# Autodesk Inventor assembly: Cockpit
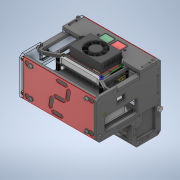
[picture p0: Inventor's stored thumbnail of the model, 180x180]
Saved by Autodesk Inventor 2022.3 (Build 263350000, 350)
## iProperties
Created: 2022-04-25
Part Number: Cockpit
Document SubType Name: Assembly
Designer: Masato Kubotera
Author: Masato Kubotera
## Documents named in this file (26)
- C:\Users\Masato\Documents\Inventor\Inventor for CIT Brains\SUSTAINA-OP - Cockpit mate\UpperBody\Cockpit\Cockpit.iam
- C:\Users\Masato\Documents\Inventor\Inventor for CIT Brains\SUSTAINA-OP - Cockpit mate\UpperBody\Cockpit\Cockpit_side_frame_MIR.ipt
- C:\Users\Masato\Documents\Inventor\Inventor for CIT Brains\SUSTAINA-OP - Cockpit mate\UpperBody\Cockpit\Cockpit_circuit_board_frame.ipt
- C:\Users\Masato\Documents\Inventor\Inventor for CIT Brains\SUSTAINA-OP - Cockpit mate\UpperBody\Cockpit\Cockpit_battery_back_door.ipt
- C:\Users\Masato\Documents\Inventor\Inventor for CIT Brains\SUSTAINA-OP - Cockpit mate\UpperBody\Cockpit\Cockpit_side_frame.ipt
- C:\Users\Masato\Documents\Inventor\Inventor for CIT Brains\SUSTAINA-OP - Cockpit mate\ReadyMade\InsertNut\IRU-304S.ipt
- C:\Users\Masato\Documents\Inventor\Inventor for CIT Brains\SUSTAINA-OP - Cockpit mate\ReadyMade\InsertNut\UD-43040.ipt
- C:\Users\Masato\Documents\Inventor\Inventor for CIT Brains\SUSTAINA-OP - Cockpit mate\ReadyMade\Neodymium_magnet_Phi3_T3.ipt
- C:\Users\Masato\Documents\Inventor\Inventor for CIT Brains\SUSTAINA-OP - Cockpit mate\UpperBody\Cockpit\Cockpit_front_frame_cloth.ipt
- C:\Users\Masato\Documents\Inventor\Inventor for CIT Brains\SUSTAINA-OP - Cockpit mate\UpperBody\Cockpit\Cockpit_back_frame_cloth.ipt
- C:\Users\Masato\Documents\Inventor\Inventor for CIT Brains\SUSTAINA-OP - Cockpit mate\ElectronicComponents\Board_designed_for_SUSTAINA-OP\SUSTAINA-Core-Board.ipt
- C:\Users\Masato\Documents\Inventor\Inventor for CIT Brains\SUSTAINA-OP - Cockpit mate\UpperBody\Cockpit\MainBoard_cover.ipt
- C:\Users\Masato\Documents\Inventor\Inventor for CIT Brains\SUSTAINA-OP - Cockpit mate\ReadyMade\Battery\HP-G830C2800S3.ipt
- C:\Users\Masato\Documents\Inventor\Inventor for CIT Brains\SUSTAINA-OP - Cockpit mate\ReadyMade\Screw\UC-0306.ipt
- C:\Users\Masato\Documents\Inventor\Inventor for CIT Brains\SUSTAINA-OP - Cockpit mate\ReadyMade\Screw\UC-0308.ipt
- C:\Users\Masato\Documents\Inventor\Inventor for CIT Brains\SUSTAINA-OP - Cockpit mate\ElectronicComponents\Board_designed_for_SUSTAINA-OP\Control-Buttons-Module.ipt
- C:\Users\Masato\Documents\Inventor\Inventor for CIT Brains\SUSTAINA-OP - Cockpit mate\ReadyMade\Screw\SPNFL-BRN-M3-10.ipt
- C:\Users\Masato\Documents\Inventor\Inventor for CIT Brains\SUSTAINA-OP - Cockpit mate\UpperBody\Cockpit\Cockpit_carrier_board_frame.iam
- C:\Users\Masato\Documents\Inventor\Inventor for CIT Brains\SUSTAINA-OP - Cockpit mate\UpperBody\Cockpit\Cockpit_top_frame.iam
- C:\Users\Masato\Documents\Inventor\Inventor for CIT Brains\SUSTAINA-OP - Cockpit mate\ElectronicComponents\SingleBoardComputerUnit.iam
- C:\Users\Masato\Documents\Inventor\Inventor for CIT Brains\SUSTAINA-OP - Cockpit mate\UpperBody\Cockpit\Cockpit_from_frame.iam
- C:\Users\Masato\Documents\Inventor\Inventor for CIT Brains\SUSTAINA-OP - Cockpit mate\ReadyMade\Bush\L3040-8110TB.ipt
- C:\Users\Masato\Documents\Inventor\Inventor for CIT Brains\SUSTAINA-OP - Cockpit mate\UpperBody\Cockpit\Cockpit_back_frame.iam
- C:\Users\Masato\Documents\Inventor\Inventor for CIT Brains\SUSTAINA-OP - Cockpit mate\ReadyMade\Screw\UC-2610.ipt
- C:\Users\Masato\Documents\Inventor\Inventor for CIT Brains\SUSTAINA-OP - Cockpit mate\ReadyMade\Spacer\BRU-305.ipt
- C:\Users\Masato\Documents\Inventor\Inventor for CIT Brains\SUSTAINA-OP - Cockpit mate\UpperBody\Cockpit\Cockpit_battery_frame.iam
## Components (88 placed, 25 different names)
1. SUSTAINA-Core-Board:1 — 挿入:63, 挿入:64, 挿入:65, 挿入:66, 挿入:95, 挿入:96, 挿入:166, 挿入:167
2. Control-Buttons-Module:1 — 挿入:105, 挿入:106, 挿入:138, 挿入:139
3. Cockpit_carrier_board_frame:1 [sub-assembly] — 挿入:140, 挿入:141, 挿入:144, 挿入:145, 挿入:149
4. Cockpit_carrier_board_frame:2 [sub-assembly] — 挿入:142, 挿入:143, 挿入:146, 挿入:147
5. Cockpit_top_frame:1 [sub-assembly] — 挿入:138, 挿入:139, 挿入:150, 挿入:151, 挿入:152, 挿入:153
6. SingleBoardComputerUnit:1 [sub-assembly] — 挿入:140, 挿入:141, 挿入:142, 挿入:143
7. UC-0308:13 — 挿入:146
8. UC-0308:14 — 挿入:147
9. Cockpit_from_frame:1 [sub-assembly] — 挿入:154, 挿入:155, 挿入:156, 挿入:157, 挿入:158, 挿入:159, 挿入:165
10. L3040-8110TB:1 — 挿入:156, 挿入:160, 挿入:164
11. L3040-8110TB:2 — 挿入:157, 挿入:161
12. L3040-8110TB:3 — 挿入:158, 挿入:162
13. L3040-8110TB:4 — 挿入:159, 挿入:163
14. UC-0306:25 — 挿入:160
15. UC-0306:26 — 挿入:161
16. UC-0306:27 — 挿入:162
17. UC-0306:28 — 挿入:163
18. UC-0308:15 — 挿入:166
19. UC-0308:16 — 挿入:167
20. Cockpit_back_frame:1 [sub-assembly] — 挿入:168, 挿入:169, 挿入:174, 挿入:175, 挿入:176, 挿入:177, 挿入:180, 挿入:181
21. L3040-8110TB:5 — 挿入:174, 挿入:178
22. UC-0306:29
23. L3040-8110TB:6 — 挿入:175, 挿入:179
24. UC-0306:30
25. L3040-8110TB:7 — 挿入:176
26. UC-0306:31
27. L3040-8110TB:8 — 挿入:177
28. UC-0306:32
29. UC-2610:1 — 挿入:180
30. UC-2610:2 — 挿入:181
31. BRU-305:1 — 挿入:182
32. BRU-305:2 — 挿入:183
33. Cockpit_battery_frame:1 [sub-assembly] — 挿入:184, 角度:4
34. Cockpit_battery_frame:2 [sub-assembly] — 挿入:185, 角度:5
35. Cockpit_side_frame_MIR:1 — 挿入:12, 挿入:23, 挿入:42, 挿入:46, 挿入:47, 挿入:48, 挿入:75, 挿入:77, 挿入:79, 挿入:80, 挿入:81, 挿入:82, 挿入:134, 挿入:137, 挿入:183
36. Cockpit_circuit_board_frame:1 — メイト:3, メイト:4, フラッシュ:8, 挿入:55, 挿入:56, 挿入:57, 挿入:58
37. Cockpit_battery_back_door:1 — 挿入:41, 挿入:42, 挿入:49, 挿入:50, 挿入:51, 挿入:52, 挿入:53, 挿入:54, 角度:3
38. Cockpit_side_frame:1 — フラッシュ:1, フラッシュ:2, フラッシュ:3, 挿入:10, 挿入:21, 挿入:41, 挿入:43, 挿入:44, 挿入:45, メイト:3, メイト:4, フラッシュ:8, 挿入:67, 挿入:68, 挿入:69, 挿入:71, 挿入:72, 挿入:73, 挿入:74, 挿入:133, 角度:3, 挿入:149, 挿入:154, 挿入:155, 挿入:168, 挿入:169, 挿入:182, 挿入:184, 角度:4, 挿入:185, 角度:5
39. Cockpit_front_frame_cloth:1 — 挿入:164, 挿入:165
40. Cockpit_back_frame_cloth:1 — 挿入:178, 挿入:179
41. MainBoard_cover:1 — 挿入:59, 挿入:60, 挿入:61, 挿入:62, 挿入:63, 挿入:64, 挿入:65, 挿入:66
42. UD-43040:1 — 挿入:21
43. UD-43040:3 — 挿入:23
44. UD-43040:5 — 挿入:55, 挿入:59
45. UD-43040:6 — 挿入:56, 挿入:60
46. UD-43040:7 — 挿入:57, 挿入:61
47. UD-43040:8 — 挿入:58, 挿入:62
48. UD-43040:11 — 挿入:133, 挿入:135
49. UD-43040:12 — 挿入:134, 挿入:136
50. HP-G830C2800S3:1
51. IRU-304S:10 — 挿入:10, 挿入:152
52. IRU-304S:12 — 挿入:12, 挿入:153
53. Neodymium_magnet_Phi3_T3:1 — 挿入:43
54. Neodymium_magnet_Phi3_T3:2 — 挿入:44
55. Neodymium_magnet_Phi3_T3:3 — 挿入:45
56. Neodymium_magnet_Phi3_T3:4 — 挿入:46
57. Neodymium_magnet_Phi3_T3:5 — 挿入:47
58. Neodymium_magnet_Phi3_T3:6 — 挿入:48
59. Neodymium_magnet_Phi3_T3:7 — 挿入:49
60. Neodymium_magnet_Phi3_T3:8 — 挿入:50
61. Neodymium_magnet_Phi3_T3:9 — 挿入:51
62. Neodymium_magnet_Phi3_T3:10 — 挿入:52
63. Neodymium_magnet_Phi3_T3:11 — 挿入:53
64. Neodymium_magnet_Phi3_T3:12 — 挿入:54
65. SPNFL-BRN-M3-10:2 — 挿入:136
66. SPNFL-BRN-M3-10:1 — 挿入:135
67. UC-0306:1 — 挿入:67
68. UC-0306:2 — 挿入:68
69. UC-0306:3 — 挿入:69
70. UC-0306:5 — 挿入:71
71. UC-0306:6 — 挿入:72
72. UC-0306:7 — 挿入:73
73. UC-0306:8 — 挿入:74
74. UC-0306:9 — 挿入:75
75. UC-0306:10 — 挿入:137
76. UC-0306:11 — 挿入:77
77. UC-0306:13 — 挿入:79
78. UC-0306:14 — 挿入:80
79. UC-0306:15 — 挿入:81
80. UC-0306:16 — 挿入:82
81. UC-0306:17 — 挿入:105
82. UC-0306:18 — 挿入:106
83. UC-0308:1 — 挿入:144
84. UC-0308:2 — 挿入:145
85. UC-0308:7 — 挿入:95
86. UC-0308:8 — 挿入:96
87. UC-0308:10 — 挿入:150
88. UC-0308:12 — 挿入:151
## Relationships (108: Insert 99, Flush 4, Angle 3, Mate 2)
- フラッシュ:1 [Flush]: Cockpit_side_frame:1
- フラッシュ:2 [Flush] (67.5 mm): Cockpit_side_frame:1
- フラッシュ:3 [Flush]: Cockpit_side_frame:1
- 挿入:10 [Insert]: Cockpit_side_frame:1 ↔ IRU-304S:10
- 挿入:12 [Insert]: Cockpit_side_frame_MIR:1 ↔ IRU-304S:12
- 挿入:21 [Insert]: Cockpit_side_frame:1 ↔ UD-43040:1
- 挿入:23 [Insert]: Cockpit_side_frame_MIR:1 ↔ UD-43040:3
- 挿入:41 [Insert]: Cockpit_battery_back_door:1 ↔ Cockpit_side_frame:1
- 挿入:42 [Insert]: Cockpit_side_frame_MIR:1 ↔ Cockpit_battery_back_door:1
- 挿入:43 [Insert]: Cockpit_side_frame:1 ↔ Neodymium_magnet_Phi3_T3:1
- 挿入:44 [Insert]: Cockpit_side_frame:1 ↔ Neodymium_magnet_Phi3_T3:2
- 挿入:45 [Insert]: Cockpit_side_frame:1 ↔ Neodymium_magnet_Phi3_T3:3
- 挿入:46 [Insert]: Cockpit_side_frame_MIR:1 ↔ Neodymium_magnet_Phi3_T3:4
- 挿入:47 [Insert]: Cockpit_side_frame_MIR:1 ↔ Neodymium_magnet_Phi3_T3:5
- 挿入:48 [Insert]: Cockpit_side_frame_MIR:1 ↔ Neodymium_magnet_Phi3_T3:6
- 挿入:49 [Insert]: Cockpit_battery_back_door:1 ↔ Neodymium_magnet_Phi3_T3:7
- 挿入:50 [Insert]: Cockpit_battery_back_door:1 ↔ Neodymium_magnet_Phi3_T3:8
- 挿入:51 [Insert]: Cockpit_battery_back_door:1 ↔ Neodymium_magnet_Phi3_T3:9
- 挿入:52 [Insert]: Cockpit_battery_back_door:1 ↔ Neodymium_magnet_Phi3_T3:10
- 挿入:53 [Insert]: Cockpit_battery_back_door:1 ↔ Neodymium_magnet_Phi3_T3:11
- 挿入:54 [Insert]: Cockpit_battery_back_door:1 ↔ Neodymium_magnet_Phi3_T3:12
- メイト:3 [Mate] (0.05 mm): Cockpit_circuit_board_frame:1 ↔ Cockpit_side_frame:1
- メイト:4 [Mate] (0.05 mm): Cockpit_circuit_board_frame:1 ↔ Cockpit_side_frame:1
- フラッシュ:8 [Flush]: Cockpit_circuit_board_frame:1 ↔ Cockpit_side_frame:1
- 挿入:55 [Insert]: Cockpit_circuit_board_frame:1 ↔ UD-43040:5
- 挿入:56 [Insert]: Cockpit_circuit_board_frame:1 ↔ UD-43040:6
- 挿入:57 [Insert]: Cockpit_circuit_board_frame:1 ↔ UD-43040:7
- 挿入:58 [Insert]: Cockpit_circuit_board_frame:1 ↔ UD-43040:8
- 挿入:59 [Insert]: MainBoard_cover:1 ↔ UD-43040:5
- 挿入:60 [Insert]: MainBoard_cover:1 ↔ UD-43040:6
- 挿入:61 [Insert]: MainBoard_cover:1 ↔ UD-43040:7
- 挿入:62 [Insert]: MainBoard_cover:1 ↔ UD-43040:8
- 挿入:63 [Insert]: SUSTAINA-Core-Board:1 ↔ MainBoard_cover:1
- 挿入:64 [Insert]: SUSTAINA-Core-Board:1 ↔ MainBoard_cover:1
- 挿入:65 [Insert]: SUSTAINA-Core-Board:1 ↔ MainBoard_cover:1
- 挿入:66 [Insert]: SUSTAINA-Core-Board:1 ↔ MainBoard_cover:1
- 挿入:67 [Insert]: Cockpit_side_frame:1 ↔ UC-0306:1
- 挿入:68 [Insert]: Cockpit_side_frame:1 ↔ UC-0306:2
- 挿入:69 [Insert]: Cockpit_side_frame:1 ↔ UC-0306:3
- 挿入:71 [Insert]: Cockpit_side_frame:1 ↔ UC-0306:5
- 挿入:72 [Insert]: Cockpit_side_frame:1 ↔ UC-0306:6
- 挿入:73 [Insert]: Cockpit_side_frame:1 ↔ UC-0306:7
- 挿入:74 [Insert]: Cockpit_side_frame:1 ↔ UC-0306:8
- 挿入:75 [Insert]: Cockpit_side_frame_MIR:1 ↔ UC-0306:9
- 挿入:77 [Insert]: Cockpit_side_frame_MIR:1 ↔ UC-0306:11
- 挿入:79 [Insert]: Cockpit_side_frame_MIR:1 ↔ UC-0306:13
- 挿入:80 [Insert]: Cockpit_side_frame_MIR:1 ↔ UC-0306:14
- 挿入:81 [Insert]: Cockpit_side_frame_MIR:1 ↔ UC-0306:15
- 挿入:82 [Insert]: Cockpit_side_frame_MIR:1 ↔ UC-0306:16
- 挿入:95 [Insert]: SUSTAINA-Core-Board:1 ↔ UC-0308:7
- 挿入:96 [Insert]: SUSTAINA-Core-Board:1 ↔ UC-0308:8
- 挿入:105 [Insert]: Control-Buttons-Module:1 ↔ UC-0306:17
- 挿入:106 [Insert]: Control-Buttons-Module:1 ↔ UC-0306:18
- 挿入:133 [Insert]: Cockpit_side_frame:1 ↔ UD-43040:11
- 挿入:134 [Insert]: Cockpit_side_frame_MIR:1 ↔ UD-43040:12
- 挿入:135 [Insert]: UD-43040:11 ↔ SPNFL-BRN-M3-10:1
- 挿入:136 [Insert]: UD-43040:12 ↔ SPNFL-BRN-M3-10:2
- 角度:3 [Angle] (0 deg): Cockpit_battery_back_door:1 ↔ Cockpit_side_frame:1
- 挿入:137 [Insert]: Cockpit_side_frame_MIR:1 ↔ UC-0306:10
- 挿入:138 [Insert]: Control-Buttons-Module:1 ↔ Cockpit_top_frame:1
- 挿入:139 [Insert]: Control-Buttons-Module:1 ↔ Cockpit_top_frame:1
- 挿入:140 [Insert]: Cockpit_carrier_board_frame:1 ↔ SingleBoardComputerUnit:1
- 挿入:141 [Insert]: Cockpit_carrier_board_frame:1 ↔ SingleBoardComputerUnit:1
- 挿入:142 [Insert]: Cockpit_carrier_board_frame:2 ↔ SingleBoardComputerUnit:1
- 挿入:143 [Insert]: Cockpit_carrier_board_frame:2 ↔ SingleBoardComputerUnit:1
- 挿入:144 [Insert]: Cockpit_carrier_board_frame:1 ↔ UC-0308:1
- 挿入:145 [Insert]: Cockpit_carrier_board_frame:1 ↔ UC-0308:2
- 挿入:146 [Insert]: Cockpit_carrier_board_frame:2 ↔ UC-0308:13
- 挿入:147 [Insert]: Cockpit_carrier_board_frame:2 ↔ UC-0308:14
- 挿入:149 [Insert]: Cockpit_carrier_board_frame:1 ↔ Cockpit_side_frame:1
- 挿入:150 [Insert]: Cockpit_top_frame:1 ↔ UC-0308:10
- 挿入:151 [Insert]: Cockpit_top_frame:1 ↔ UC-0308:12
- 挿入:152 [Insert]: Cockpit_top_frame:1 ↔ IRU-304S:10
- 挿入:153 [Insert]: Cockpit_top_frame:1 ↔ IRU-304S:12
- 挿入:154 [Insert]: Cockpit_from_frame:1 ↔ Cockpit_side_frame:1
- 挿入:155 [Insert]: Cockpit_from_frame:1 ↔ Cockpit_side_frame:1
- 挿入:156 [Insert]: Cockpit_from_frame:1 ↔ L3040-8110TB:1
- 挿入:157 [Insert]: Cockpit_from_frame:1 ↔ L3040-8110TB:2
- 挿入:158 [Insert]: Cockpit_from_frame:1 ↔ L3040-8110TB:3
- 挿入:159 [Insert]: Cockpit_from_frame:1 ↔ L3040-8110TB:4
- 挿入:160 [Insert]: L3040-8110TB:1 ↔ UC-0306:25
- 挿入:161 [Insert]: L3040-8110TB:2 ↔ UC-0306:26
- 挿入:162 [Insert]: L3040-8110TB:3 ↔ UC-0306:27
- 挿入:163 [Insert]: L3040-8110TB:4 ↔ UC-0306:28
- 挿入:164 [Insert]: L3040-8110TB:1 ↔ Cockpit_front_frame_cloth:1
- 挿入:165 [Insert]: Cockpit_from_frame:1 ↔ Cockpit_front_frame_cloth:1
- 挿入:166 [Insert]: SUSTAINA-Core-Board:1 ↔ UC-0308:15
- 挿入:167 [Insert]: SUSTAINA-Core-Board:1 ↔ UC-0308:16
- 挿入:168 [Insert]: Cockpit_back_frame:1 ↔ Cockpit_side_frame:1
- 挿入:169 [Insert]: Cockpit_back_frame:1 ↔ Cockpit_side_frame:1
- [Insert]: L3040-8110TB:5 ↔ UC-0306:29
- [Insert]: L3040-8110TB:6 ↔ UC-0306:30
- [Insert]: L3040-8110TB:7 ↔ UC-0306:31
- [Insert]: L3040-8110TB:8 ↔ UC-0306:32
- 挿入:174 [Insert]: Cockpit_back_frame:1 ↔ L3040-8110TB:5
- 挿入:175 [Insert]: Cockpit_back_frame:1 ↔ L3040-8110TB:6
- 挿入:176 [Insert]: Cockpit_back_frame:1 ↔ L3040-8110TB:7
- 挿入:177 [Insert]: Cockpit_back_frame:1 ↔ L3040-8110TB:8
- 挿入:178 [Insert]: L3040-8110TB:5 ↔ Cockpit_back_frame_cloth:1
- 挿入:179 [Insert]: L3040-8110TB:6 ↔ Cockpit_back_frame_cloth:1
- 挿入:180 [Insert]: Cockpit_back_frame:1 ↔ UC-2610:1
- 挿入:181 [Insert]: Cockpit_back_frame:1 ↔ UC-2610:2
- 挿入:182 [Insert]: BRU-305:1 ↔ Cockpit_side_frame:1
- 挿入:183 [Insert]: BRU-305:2 ↔ Cockpit_side_frame_MIR:1
- 挿入:184 [Insert]: Cockpit_battery_frame:1 ↔ Cockpit_side_frame:1
- 角度:4 [Angle] (0 deg): Cockpit_battery_frame:1 ↔ Cockpit_side_frame:1
- 挿入:185 [Insert]: Cockpit_battery_frame:2 ↔ Cockpit_side_frame:1
- 角度:5 [Angle] (0 deg): Cockpit_battery_frame:2 ↔ Cockpit_side_frame:1
## Named parameters: d215_d205 = 0 mm, d216_d205 = 0 mm, d217_d205 = 0 mm, d218_d205 = 0 mm
